# Autodesk Inventor assembly: Manfrotto - 494RC2 Head Assy
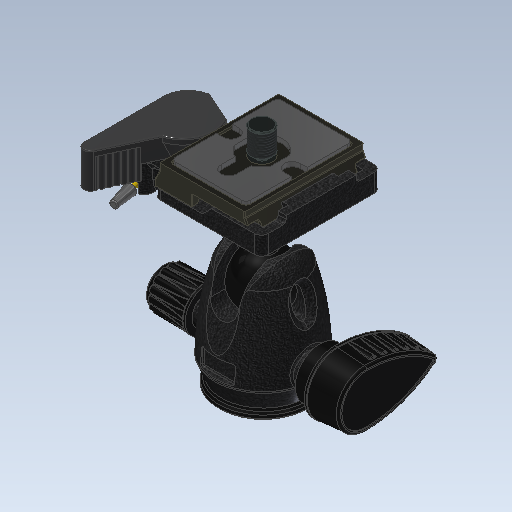
[picture p0: Inventor's stored thumbnail of the model, 512x512]
Saved by Autodesk Inventor 2020 (Build 240168000, 168)
## iProperties
Created: 2012-10-13
Part Number: Manfrotto - 494RC2 Head Assy
Document SubType Name: Assembly
Designer: Lance
Mass: 790.219 g
Surface Area: 506.772 cm^2
Volume: 120.63 cm^3
Density: 6.55078 g/cm^3
Author: Lance
## Documents named in this file (12)
- C:\Users\Hesekiel\Desktop\Equatorial-Mount-MUM\Mechanika\Mechanizm elewacji Filip\CAD\manfrotto-494rc2-tripod-head.snapshot.1\Manfrotto 494RC2 - Tripod Head\Manfrotto - 494RC2 Head Assy.iam
- C:\Users\Hesekiel\Desktop\Equatorial-Mount-MUM\Mechanika\Mechanizm elewacji Filip\CAD\manfrotto-494rc2-tripod-head.snapshot.1\Manfrotto 494RC2 - Tripod Head\Base Casting.ipt
- C:\Users\Hesekiel\Desktop\Equatorial-Mount-MUM\Mechanika\Mechanizm elewacji Filip\CAD\manfrotto-494rc2-tripod-head.snapshot.1\Manfrotto 494RC2 - Tripod Head\Base Plate.ipt
- C:\Users\Hesekiel\Desktop\Equatorial-Mount-MUM\Mechanika\Mechanizm elewacji Filip\CAD\manfrotto-494rc2-tripod-head.snapshot.1\Manfrotto 494RC2 - Tripod Head\Mount Casting.ipt
- C:\Users\Hesekiel\Desktop\Equatorial-Mount-MUM\Mechanika\Mechanizm elewacji Filip\CAD\manfrotto-494rc2-tripod-head.snapshot.1\Manfrotto 494RC2 - Tripod Head\Ball Joint.ipt
- C:\Users\Hesekiel\Desktop\Equatorial-Mount-MUM\Mechanika\Mechanizm elewacji Filip\CAD\manfrotto-494rc2-tripod-head.snapshot.1\Manfrotto 494RC2 - Tripod Head\ISO 10642 - M5 x  16 (Stainless Steel).ipt
- C:\Users\Hesekiel\Desktop\Equatorial-Mount-MUM\Mechanika\Mechanizm elewacji Filip\CAD\manfrotto-494rc2-tripod-head.snapshot.1\Manfrotto 494RC2 - Tripod Head\Quick Release Assy.iam
- C:\Users\Hesekiel\Desktop\Equatorial-Mount-MUM\Mechanika\Mechanizm elewacji Filip\CAD\manfrotto-494rc2-tripod-head.snapshot.1\Manfrotto 494RC2 - Tripod Head\Quick Release Catch.ipt
- C:\Users\Hesekiel\Desktop\Equatorial-Mount-MUM\Mechanika\Mechanizm elewacji Filip\CAD\manfrotto-494rc2-tripod-head.snapshot.1\Manfrotto 494RC2 - Tripod Head\Friction Knob.ipt
- C:\Users\Hesekiel\Desktop\Equatorial-Mount-MUM\Mechanika\Mechanizm elewacji Filip\CAD\manfrotto-494rc2-tripod-head.snapshot.1\Manfrotto 494RC2 - Tripod Head\Locking Knob.ipt
- C:\Users\Hesekiel\Desktop\Equatorial-Mount-MUM\Mechanika\Mechanizm elewacji Filip\CAD\manfrotto-494rc2-tripod-head.snapshot.1\Manfrotto 494RC2 - Tripod Head\Manfrotto Logo 01.iam
- C:\Users\Hesekiel\Desktop\Equatorial-Mount-MUM\Mechanika\Mechanizm elewacji Filip\CAD\manfrotto-494rc2-tripod-head.snapshot.1\Manfrotto 494RC2 - Tripod Head\Locking Pin Assy.iam
## Components (11 placed, 11 different names)
1. Base Casting:1 — Flush:1, Mate:1, Flush:2, Mate:2, Flush:3, Flush:4, Mate:7, Angle:3, Mate:9, Mate:10, Mate:11, Angle:4, Insert:3, Angle:5
2. Base Plate:1 — Flush:1, Mate:1, Flush:2
3. Mount Casting:1 — Insert:1, Flush:5, Mate:3, Mate:4, Angle:1, Mate:5, Mate:6, Tangent:1, Insert:2, Insert:4, Angle:6
4. Ball Joint:1 — Mate:2, Flush:3, Flush:4, Insert:1, Flush:5
5. ISO 10642 M5 x  16:2 — Mate:3, Mate:4, Angle:1
6. Quick Release Assy:1 [sub-assembly] — Mate:5, Mate:6, Tangent:1, Angle:2
7. Quick Release Catch:1 — Insert:2, Angle:2
8. Friction Knob:1 — Mate:7, Angle:3, Mate:9
9. Locking Knob:1 — Mate:10, Mate:11, Angle:4
10. Manfrotto Logo 01:1 [sub-assembly] — Insert:3, Angle:5
11. Locking Pin Assy:1 [sub-assembly] — Insert:4, Angle:6
## Relationships (26: Mate 10, Angle 6, Flush 5, Insert 4, Tangent 1)
- Flush:1 (4 mm): Base Casting:1 ↔ Base Plate:1
- Mate:1: Base Casting:1 ↔ Base Plate:1
- Flush:2: Base Casting:1 ↔ Base Plate:1
- Mate:2: Base Casting:1 ↔ Ball Joint:1
- Flush:3: Base Casting:1 ↔ Ball Joint:1
- Flush:4: Base Casting:1 ↔ Ball Joint:1
- Insert:1: Mount Casting:1 ↔ Ball Joint:1
- Flush:5: Mount Casting:1 ↔ Ball Joint:1
- Mate:3: Mount Casting:1 ↔ ISO 10642 M5 x  16:2
- Mate:4: Mount Casting:1 ↔ ISO 10642 M5 x  16:2
- Angle:1 (0 deg): Mount Casting:1 ↔ ISO 10642 M5 x  16:2
- Mate:5: Mount Casting:1 ↔ Quick Release Assy:1
- Mate:6: Mount Casting:1 ↔ Quick Release Assy:1
- Tangent:1: Mount Casting:1 ↔ Quick Release Assy:1
- Insert:2: Mount Casting:1 ↔ Quick Release Catch:1
- Angle:2 (0 deg): Quick Release Assy:1 ↔ Quick Release Catch:1
- Mate:7: Base Casting:1 ↔ Friction Knob:1
- Angle:3 (0 deg): Base Casting:1 ↔ Friction Knob:1
- Mate:9 (25 mm): Base Casting:1 ↔ Friction Knob:1
- Mate:10: Base Casting:1 ↔ Locking Knob:1
- Mate:11 (25 mm): Base Casting:1 ↔ Locking Knob:1
- Angle:4 (180 deg): Base Casting:1 ↔ Locking Knob:1
- Insert:3: Base Casting:1 ↔ Manfrotto Logo 01:1
- Angle:5 (180 deg): Base Casting:1 ↔ Manfrotto Logo 01:1
- Insert:4: Mount Casting:1 ↔ Locking Pin Assy:1
- Angle:6 (13 deg): Mount Casting:1 ↔ Locking Pin Assy:1
